# Autodesk Inventor assembly: единое крепление
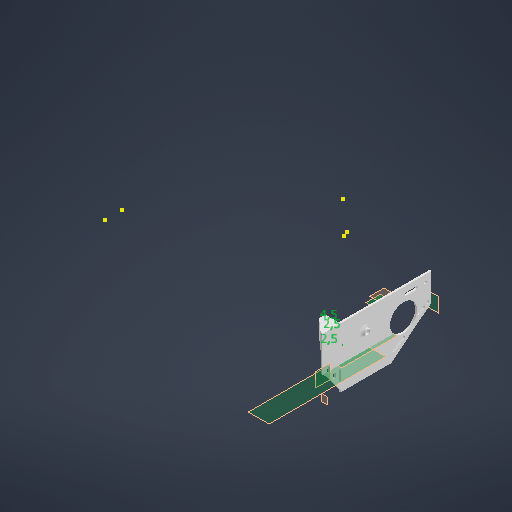
[picture p0: Inventor's stored thumbnail of the model, 512x512]
Saved by Autodesk Inventor 2025 (Build 290162000, 162)
## iProperties
Created: 2024-09-25
Part Number: единое крепление
Document SubType Name: Assembly
Designer: GameHD
Author: GameHD
## Documents named in this file (5)
- C:\Users\Phantom\Desktop\Phantom16950\единое крепление.iam
- C:\Users\Phantom\Desktop\Phantom16950\крепл для колёс.ipt
- C:\Users\Phantom\Desktop\Phantom16950\крепл для колёс. 2 часть.ipt
- C:\Users\Phantom\Desktop\Phantom16950\крепл для колёс встав часть. вторая часть.ipt
- C:\Users\Phantom\Desktop\Phantom16950\крепл для колёс встав часть.ipt
## Components (4 placed, 4 different names)
1. крепл для колёс:1 — Совмещение:4, Заподлицо:5, Совмещение:5, Заподлицо:7, Заподлицо:9, Совмещение:8, Совмещение:9, Заподлицо:11, Заподлицо:12, Заподлицо:13, Совмещение:11
2. крепл для колёс. 2 часть:1 — Совмещение:4, Заподлицо:5, Совмещение:6, Заподлицо:8, Заподлицо:10, Совмещение:10, Заподлицо:13
3. крепл для колёс встав часть. вторая часть:1 — Совмещение:6, Заподлицо:6, Совмещение:7, Заподлицо:7, Заподлицо:8, Заподлицо:10, Совмещение:10, Заподлицо:12
4. крепл для колёс встав часть:1 — Совмещение:5, Заподлицо:6, Совмещение:7, Совмещение:8, Совмещение:9, Заподлицо:11, Совмещение:11
## Relationships (17: Flush 9, Mate 8)
- Совмещение:4 [Mate]: крепл для колёс:1 ↔ крепл для колёс. 2 часть:1
- Заподлицо:5 [Flush]: крепл для колёс:1 ↔ крепл для колёс. 2 часть:1
- Совмещение:5 [Mate]: крепл для колёс:1 ↔ крепл для колёс встав часть:1
- Совмещение:6 [Mate]: крепл для колёс. 2 часть:1 ↔ крепл для колёс встав часть. вторая часть:1
- Заподлицо:6 [Flush]: крепл для колёс встав часть. вторая часть:1 ↔ крепл для колёс встав часть:1
- Совмещение:7 [Mate]: крепл для колёс встав часть. вторая часть:1 ↔ крепл для колёс встав часть:1
- Заподлицо:7 [Flush]: крепл для колёс:1 ↔ крепл для колёс встав часть. вторая часть:1
- Заподлицо:8 [Flush]: крепл для колёс. 2 часть:1 ↔ крепл для колёс встав часть. вторая часть:1
- Заподлицо:9 [Flush]: крепл для колёс:1
- Совмещение:8 [Mate]: крепл для колёс:1 ↔ крепл для колёс встав часть:1
- Заподлицо:10 [Flush]: крепл для колёс. 2 часть:1 ↔ крепл для колёс встав часть. вторая часть:1
- Совмещение:9 [Mate]: крепл для колёс:1 ↔ крепл для колёс встав часть:1
- Совмещение:10 [Mate]: крепл для колёс. 2 часть:1 ↔ крепл для колёс встав часть. вторая часть:1
- Заподлицо:11 [Flush]: крепл для колёс:1 ↔ крепл для колёс встав часть:1
- Заподлицо:12 [Flush]: крепл для колёс:1 ↔ крепл для колёс встав часть. вторая часть:1
- Заподлицо:13 [Flush]: крепл для колёс:1 ↔ крепл для колёс. 2 часть:1
- Совмещение:11 [Mate]: крепл для колёс:1 ↔ крепл для колёс встав часть:1
